# Autodesk Inventor assembly: CA[FD1][Manufacture Assambly]
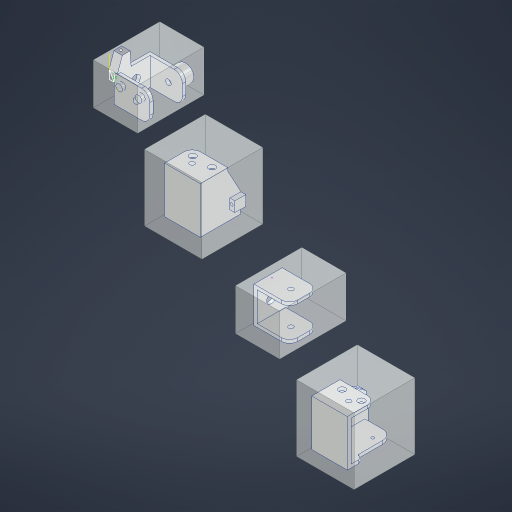
[picture p0: Inventor's stored thumbnail of the model, 512x512]
Saved by Autodesk Inventor 2024 (Build 280153000, 153)
## iProperties
Created: 2023-06-19
Part Number: CA[FD1][Manufacture Assambly]
Document SubType Name: Assembly
Designer: juanj
Author: juanj
## Documents named in this file (7)
- C:\Users\juanj\Documents\Documentos\Unisabana\Shell\C23[1stD]\CA[FD1][Manufacture Assambly].iam
- C:\Users\juanj\Documents\Documentos\Unisabana\Shell\C23[1stD]\Upper Right Building Block.ipt
- C:\Users\juanj\Documents\Documentos\Unisabana\Shell\C23[1stD]\Down Right Building Block.ipt
- C:\Users\juanj\Documents\Documentos\Unisabana\Shell\C23[1stD]\C23[L][FD1].ipt
- C:\Users\juanj\Documents\Documentos\Unisabana\Shell\C23[1stD]\C23[R][FD1].ipt
- C:\Users\juanj\Documents\Documentos\Unisabana\Shell\C23[1stD]\DC23[L][FD1].ipt
- C:\Users\juanj\Documents\Documentos\Unisabana\Shell\C23[1stD]\DC23[R][FD1].ipt
## Components (8 placed, 8 different names)
1. Upper Right Building Block — Angle:1, Angle:5
2. Upper Left Building Block — Angle:3
3. Down Right Building Block — Angle:2
4. Down Left Building Block — Angle:4
5. C23[L][FD1]:1 — Angle:1, Angle:5
6. C23[R][FD1]:1 — Angle:3
7. DC23[L][FD1]:1 — Angle:2
8. DC23[R][FD1]:1 — Angle:4
## Relationships (5: Angle 5)
- Angle:1 (0 deg): Upper Right Building Block ↔ C23[L][FD1]:1
- Angle:2 (0 deg): Down Right Building Block ↔ DC23[L][FD1]:1
- Angle:3 (0 deg): Upper Left Building Block ↔ C23[R][FD1]:1
- Angle:4 (0 deg): Down Left Building Block ↔ DC23[R][FD1]:1
- Angle:5 (0 deg): Upper Right Building Block ↔ C23[L][FD1]:1
